# Autodesk Inventor assembly: iPadHolderAssembly
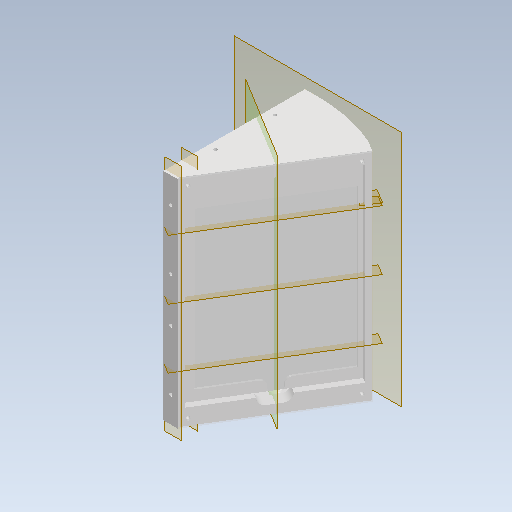
[picture p0: Inventor's stored thumbnail of the model, 512x512]
Saved by Autodesk Inventor 2021.3 (Build 253353000, 353)
## iProperties
Created: 2020-11-06
Part Number: iPadHolderAssembly
Document SubType Name: Assembly
Designer: gisen
Author: gisen
## Documents named in this file (3)
- C:\Users\gisen\GitProjects\CAD-Data\CuboidAccessories\SecurityBox\Assemblies\DisplayHolderAssembly.iam
- C:\Users\gisen\GitProjects\CAD-Data\CuboidAccessories\SecurityBox\3DPrintedParts\DisplayHolder.ipt
- C:\Users\gisen\GitProjects\CAD-Data\CuboidAccessories\SecurityBox\Plates\iPadCoverPlate.ipt
## Components (2 placed, 2 different names)
1. DisplayHolder:1 — メイト:4, メイト:5, メイト:6, メイト:9, メイト:10, フラッシュ:1
2. iPadCoverPlate:1 — メイト:9, メイト:10, フラッシュ:1
## Relationships (6: Mate 5, Flush 1)
- メイト:4 [Mate]: DisplayHolder:1
- メイト:5 [Mate]: DisplayHolder:1
- メイト:6 [Mate]: DisplayHolder:1
- メイト:9 [Mate]: DisplayHolder:1 ↔ iPadCoverPlate:1
- メイト:10 [Mate]: DisplayHolder:1 ↔ iPadCoverPlate:1
- フラッシュ:1 [Flush]: DisplayHolder:1 ↔ iPadCoverPlate:1
